# Autodesk Inventor assembly: Assembly
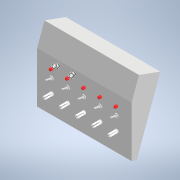
[picture p0: Inventor's stored thumbnail of the model, 180x180]
Saved by Autodesk Inventor 2021 (Build 250183000, 183)
## iProperties
Created: 2020-07-28
Part Number: Assembly
Document SubType Name: Assembly
Designer: johna
Author: johna
## Documents named in this file (12)
- C:\Users\johna\OneDrive\Desktop\Arduino-Soundboard\CAD\Assembly.iam
- C:\Users\johna\OneDrive\Desktop\Arduino-Soundboard\CAD\front.ipt
- C:\Users\johna\OneDrive\Desktop\Arduino-Soundboard\CAD\LED 5mm Red height 1-20mm\LED Heigth mm 20.0.ipt
- C:\Users\johna\OneDrive\Desktop\Arduino-Soundboard\CAD\LED 5mm Red height 1-20mm.ipt
- C:\Users\johna\OneDrive\Desktop\Arduino-Soundboard\CAD\200-MSP-1-T3-B1-M2-PE-rev2.ipt
- C:\Users\johna\OneDrive\Desktop\Arduino-Soundboard\CAD\47K Potenziometer.ipt
- C:\Users\johna\OneDrive\Desktop\Arduino-Soundboard\CAD\Arduino_Uno.ipt
- C:\Users\johna\OneDrive\Desktop\Arduino-Soundboard\CAD\side.ipt
- C:\Users\johna\OneDrive\Desktop\Arduino-Soundboard\CAD\bottom.ipt
- C:\Users\johna\OneDrive\Desktop\Arduino-Soundboard\CAD\sideWithHole.ipt
- C:\Users\johna\OneDrive\Desktop\Arduino-Soundboard\CAD\top.ipt
- C:\Users\johna\OneDrive\Desktop\Arduino-Soundboard\CAD\back.ipt
## Components (22 placed, 10 different names)
1. front:1 — Insert:1, Insert:2, Insert:3, Insert:4, Insert:5, Mate:1, Mate:2, Insert:6, Mate:3, Mate:4, Mate:5, Mate:6, Mate:7, Mate:8, Mate:9, Mate:10, Mate:11, Mate:12, Mate:13, Mate:14, Mate:20, Mate:25, Mate:26, Mate:31, Mate:33
2. LED Heigth mm 20.0:1 — Insert:5
3. LED Heigth mm 20.0:2 — Insert:1
4. LED Heigth mm 20.0:3 — Insert:2
5. LED Heigth mm 20.0:4 — Insert:3
6. LED Heigth mm 20.0:5 — Insert:4
7. 200-MSP-1-T3-B1-M2-PE-rev2:1 — Insert:6
8. 47K Potenziometer:1 — Mate:1, Mate:2
9. Arduino_Uno:1 — Mate:28, Flush:3, Mate:29
10. 47K Potenziometer:2 — Mate:3, Mate:4
11. 47K Potenziometer:3 — Mate:5, Mate:6
12. 47K Potenziometer:4 — Mate:7, Mate:8
13. 47K Potenziometer:5 — Mate:9, Mate:10
14. 200-MSP-1-T3-B1-M2-PE-rev2:2 — Mate:13
15. 200-MSP-1-T3-B1-M2-PE-rev2:3 — Mate:11
16. 200-MSP-1-T3-B1-M2-PE-rev2:4 — Mate:12
17. 200-MSP-1-T3-B1-M2-PE-rev2:5 — Mate:14
18. side:2 — Mate:20, Mate:27, Flush:1, Mate:33
19. bottom:1 — Mate:27, Flush:1, Mate:28, Flush:4
20. sideWithHole:1 — Mate:25, Mate:26, Flush:3, Mate:29, Flush:4, Mate:34, Mate:35, Flush:6
21. top:1 — Mate:31, Mate:34, Flush:5
22. back:1 — Mate:35, Flush:5, Flush:6
## Relationships (35: Mate 24, Insert 6, Flush 5)
- Insert:1: front:1 ↔ LED Heigth mm 20.0:2
- Insert:2: front:1 ↔ LED Heigth mm 20.0:3
- Insert:3: front:1 ↔ LED Heigth mm 20.0:4
- Insert:4: front:1 ↔ LED Heigth mm 20.0:5
- Insert:5: front:1 ↔ LED Heigth mm 20.0:1
- Mate:1: front:1 ↔ 47K Potenziometer:1
- Mate:2: front:1 ↔ 47K Potenziometer:1
- Insert:6: front:1 ↔ 200-MSP-1-T3-B1-M2-PE-rev2:1
- Mate:3: front:1 ↔ 47K Potenziometer:2
- Mate:4: front:1 ↔ 47K Potenziometer:2
- Mate:5: front:1 ↔ 47K Potenziometer:3
- Mate:6: front:1 ↔ 47K Potenziometer:3
- Mate:7: front:1 ↔ 47K Potenziometer:4
- Mate:8: front:1 ↔ 47K Potenziometer:4
- Mate:9: front:1 ↔ 47K Potenziometer:5
- Mate:10: front:1 ↔ 47K Potenziometer:5
- Mate:11: front:1 ↔ 200-MSP-1-T3-B1-M2-PE-rev2:3
- Mate:12: front:1 ↔ 200-MSP-1-T3-B1-M2-PE-rev2:4
- Mate:13: front:1 ↔ 200-MSP-1-T3-B1-M2-PE-rev2:2
- Mate:14: front:1 ↔ 200-MSP-1-T3-B1-M2-PE-rev2:5
- Mate:20: front:1 ↔ side:2
- Mate:25: front:1 ↔ sideWithHole:1
- Mate:26: front:1 ↔ sideWithHole:1
- Mate:27: side:2 ↔ bottom:1
- Flush:1: side:2 ↔ bottom:1
- Mate:28 (0.762 mm): Arduino_Uno:1 ↔ bottom:1
- Flush:3: Arduino_Uno:1 ↔ sideWithHole:1
- Mate:29: Arduino_Uno:1 ↔ sideWithHole:1
- Flush:4: bottom:1 ↔ sideWithHole:1
- Mate:31: front:1 ↔ top:1
- Mate:33: front:1 ↔ side:2
- Mate:34: sideWithHole:1 ↔ top:1
- Mate:35: sideWithHole:1 ↔ back:1
- Flush:5: top:1 ↔ back:1
- Flush:6: sideWithHole:1 ↔ back:1
